# Autodesk Inventor assembly: OT2-Gripper V1-1 BG
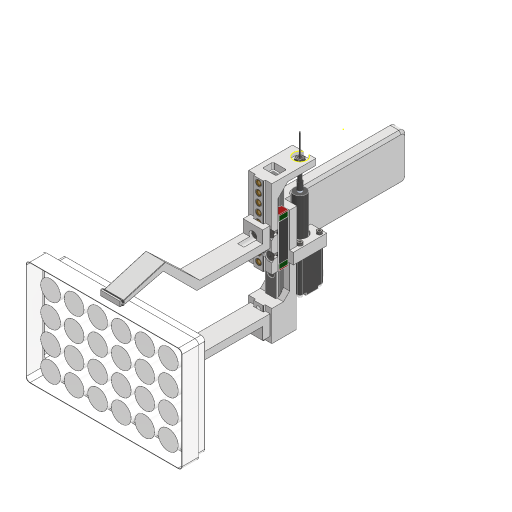
[picture p0: Inventor's stored thumbnail of the model, 512x512]
Saved by Autodesk Inventor 2024.3 (Build 283343000, 343)
## iProperties
Created: 2024-09-13
Part Number: OT2-Gripper V1-1 BG
Document SubType Name: Assembly
Designer: Martin
Author: Martin
## Documents named in this file (15)
- D:\User\Dokumente\GitHub\openUC2-OT2-PlateGripper\INVENTOR\OT2-Gripper V1-1 BG.iam
- D:\User\Dokumente\GitHub\openUC2-OT2-PlateGripper\INVENTOR\OT2-Gripper V1-1 - gripper A.ipt
- D:\User\Dokumente\GitHub\openUC2-OT2-PlateGripper\INVENTOR\OT2-Gripper V1-1 - OT2-interface adapter.ipt
- D:\User\Dokumente\GitHub\openUC2-OT2-PlateGripper\INVENTOR\OT2-Gripper V1-1 - linear adapter static.ipt
- D:\User\Dokumente\GitHub\openUC2-OT2-PlateGripper\INVENTOR\OT2-Gripper V1-1 - linear-adapter.ipt
- D:\User\Dokumente\GitHub\openUC2-OT2-PlateGripper\INVENTOR\00_Joy-IT-B20SHD4353_NEMA8_captive.ipt
- D:\User\Dokumente\GitHub\openUC2-OT2-PlateGripper\INVENTOR\Threaded Insert-Ruthex-M3.ipt
- D:\User\Dokumente\Inventor\Content Center Files\R2024\de-DE\ISO 4032(2)\ISO 4032 - M3 - ISO.ipt
- D:\User\Dokumente\GitHub\openUC2-OT2-PlateGripper\INVENTOR\Actuator_MGN-BG.iam
- D:\User\Dokumente\GitHub\openUC2-OT2-PlateGripper\INVENTOR\00_24wellplate_base_2.ipt
- D:\User\Dokumente\Inventor\Content Center Files\R2024\de-DE\ISO 7091\ISO 7091 - ST 3 - 100 HV.ipt
- D:\User\Dokumente\GitHub\openUC2-OT2-PlateGripper\INVENTOR\o-ring eg MISUMI NSF12.ipt
- D:\User\Dokumente\Inventor\Content Center Files\R2024\de-DE\ISO 4762(2)\ISO 4762 - M2 x 12ISO.ipt
- D:\User\Dokumente\Inventor\Content Center Files\R2024\de-DE\ISO 10642(1)\ISO 10642 - M3 x  8.ipt
- D:\User\Dokumente\Inventor\Content Center Files\R2024\de-DE\ISO 4762(2)\ISO 4762 - M3 x 8ISO.ipt
## Components (44 placed, 14 different names)
1. OT2-Gripper V1-1 - OT2-interface adapter:1 — Einfügen:1, Einfügen:2, Einfügen:3, Passend:1, Passend:3, Passend:9, Einfügen:27, Einfügen:28, Einfügen:29, Einfügen:30, Einfügen:31, Einfügen:32
2. OT2-Gripper V1-1 - linear adapter static:1 — Einfügen:6, Einfügen:7, Einfügen:15, Einfügen:16, Winkel:2, Winkel:3, Passend:2, Passend:8, Winkel:4, Passend:12, Passend:13
3. OT2-Gripper V1-1 - linear-adapter:1 — Einfügen:4, Einfügen:5, Einfügen:8, Einfügen:9, Einfügen:10, Einfügen:11, Einfügen:12, Einfügen:13, Einfügen:14, Passend:4, Passend:5, Passend:6, Passend:7, Passend:10, Passend:11, Passend:14, Einfügen:26
4. OT2-Gripper V1-1 - gripper A:1 — Fluchtend:1, Fluchtend:2, Passend:12, Einfügen:17, Fluchtend:4, Tangential:5, Tangential:6, Tangential:7, Tangential:8, Passend:13
5. OT2-Gripper V1-1 - gripper A:2 — Fluchtend:1, Fluchtend:2, Passend:14, Tangential:1, Tangential:2, Tangential:3, Tangential:4
6. Threaded Insert-Ruthex-M3:14 — Einfügen:29
7. Threaded Insert-Ruthex-M3:15 — Einfügen:27
8. Threaded Insert-Ruthex-M3:16 — Einfügen:28
9. o-ring eg MISUMI NSF12:1 — Tangential:5, Tangential:6, Tangential:7, Tangential:8, Tangential:9
10. o-ring eg MISUMI NSF12:2 — Tangential:1, Tangential:2, Tangential:3, Tangential:4
11. Threaded Insert-Ruthex-M3:1 — Einfügen:3
12. Threaded Insert-Ruthex-M3:2 — Einfügen:4
13. Threaded Insert-Ruthex-M3:3 — Einfügen:5
14. Threaded Insert-Ruthex-M3:4 — Einfügen:2
15. Threaded Insert-Ruthex-M3:5 — Einfügen:14
16. Threaded Insert-Ruthex-M3:6 — Einfügen:13
17. Threaded Insert-Ruthex-M3:7 — Einfügen:12
18. Threaded Insert-Ruthex-M3:8 — Einfügen:11, Einfügen:18
19. Threaded Insert-Ruthex-M3:9 — Einfügen:10
20. Threaded Insert-Ruthex-M3:10 — Einfügen:9
21. Threaded Insert-Ruthex-M3:11 — Einfügen:7
22. Threaded Insert-Ruthex-M3:12 — Einfügen:6
23. Threaded Insert-Ruthex-M3:13 — Einfügen:8
24. 00_Joy-IT-B20SHD4353_NEMA8_captive:1 — Einfügen:1, Winkel:1, Passend:11
25. Actuator_MGN-BG:1 [sub-assembly] — Passend:1, Passend:2, Passend:3, Passend:4, Passend:5, Passend:6, Passend:7, Passend:8, Winkel:4, Passend:9, Passend:10
26. ISO 4762 M2 x 12:1 — Einfügen:30
27. ISO 4762 M2 x 12:2 — Einfügen:31
28. ISO 4762 M2 x 12:3 — Einfügen:32
29. ISO 10642 M3x8:1
30. ISO 10642 M3x8:2
31. ISO 10642 M3x8:3
32. ISO 10642 M3x8:4
33. ISO 4032 M3:3 — Einfügen:25, Einfügen:26
34. ISO 7091 ST 3 - 100 HV:1 — Einfügen:25
35. ISO 4032 M3:1 — Einfügen:16, Winkel:3
36. ISO 4032 M3:2 — Einfügen:15, Winkel:2
37. ISO 4762 M3 x 8:1 — Einfügen:17
38. ISO 4762 M3 x 8:2 — Einfügen:18
39. ISO 4762 M3 x 8:3
40. ISO 4762 M3 x 8:4
41. ISO 4762 M3 x 8:5
42. ISO 4762 M3 x 8:6
43. ISO 4762 M3 x 8:7
44. 00_24wellplate_base_2:1 — Fluchtend:3, Fluchtend:4, Tangential:9
## Relationships (66: Insert 31, Mate 18, Tangent 9, Angle 4, Flush 4)
- Einfügen:1 [Insert]: OT2-Gripper V1-1 - OT2-interface adapter:1 ↔ 00_Joy-IT-B20SHD4353_NEMA8_captive:1
- Winkel:1 [Angle] (180 deg): 00_Joy-IT-B20SHD4353_NEMA8_captive:1
- Einfügen:2 [Insert]: OT2-Gripper V1-1 - OT2-interface adapter:1 ↔ Threaded Insert-Ruthex-M3:4
- Einfügen:3 [Insert]: OT2-Gripper V1-1 - OT2-interface adapter:1 ↔ Threaded Insert-Ruthex-M3:1
- Einfügen:4 [Insert]: OT2-Gripper V1-1 - linear-adapter:1 ↔ Threaded Insert-Ruthex-M3:2
- Einfügen:5 [Insert]: OT2-Gripper V1-1 - linear-adapter:1 ↔ Threaded Insert-Ruthex-M3:3
- Einfügen:6 [Insert]: OT2-Gripper V1-1 - linear adapter static:1 ↔ Threaded Insert-Ruthex-M3:12
- Einfügen:7 [Insert]: OT2-Gripper V1-1 - linear adapter static:1 ↔ Threaded Insert-Ruthex-M3:11
- Einfügen:8 [Insert]: OT2-Gripper V1-1 - linear-adapter:1 ↔ Threaded Insert-Ruthex-M3:13
- Einfügen:9 [Insert]: OT2-Gripper V1-1 - linear-adapter:1 ↔ Threaded Insert-Ruthex-M3:10
- Einfügen:10 [Insert]: OT2-Gripper V1-1 - linear-adapter:1 ↔ Threaded Insert-Ruthex-M3:9
- Einfügen:11 [Insert]: OT2-Gripper V1-1 - linear-adapter:1 ↔ Threaded Insert-Ruthex-M3:8
- Einfügen:12 [Insert]: OT2-Gripper V1-1 - linear-adapter:1 ↔ Threaded Insert-Ruthex-M3:7
- Einfügen:13 [Insert]: OT2-Gripper V1-1 - linear-adapter:1 ↔ Threaded Insert-Ruthex-M3:6
- Einfügen:14 [Insert]: OT2-Gripper V1-1 - linear-adapter:1 ↔ Threaded Insert-Ruthex-M3:5
- Einfügen:15 [Insert]: OT2-Gripper V1-1 - linear adapter static:1 ↔ ISO 4032 M3:2
- Einfügen:16 [Insert]: OT2-Gripper V1-1 - linear adapter static:1 ↔ ISO 4032 M3:1
- Winkel:2 [Angle] (0 deg): OT2-Gripper V1-1 - linear adapter static:1 ↔ ISO 4032 M3:2
- Winkel:3 [Angle] (0 deg): OT2-Gripper V1-1 - linear adapter static:1 ↔ ISO 4032 M3:1
- Passend:1 [Mate]: OT2-Gripper V1-1 - OT2-interface adapter:1 ↔ Actuator_MGN-BG:1
- Passend:2 [Mate]: OT2-Gripper V1-1 - linear adapter static:1 ↔ Actuator_MGN-BG:1
- Passend:3 [Mate]: OT2-Gripper V1-1 - OT2-interface adapter:1 ↔ Actuator_MGN-BG:1
- Passend:4 [Mate]: OT2-Gripper V1-1 - linear-adapter:1 ↔ Actuator_MGN-BG:1
- Passend:5 [Mate]: OT2-Gripper V1-1 - linear-adapter:1 ↔ Actuator_MGN-BG:1
- Passend:6 [Mate]: OT2-Gripper V1-1 - linear-adapter:1 ↔ Actuator_MGN-BG:1
- Passend:7 [Mate]: OT2-Gripper V1-1 - linear-adapter:1 ↔ Actuator_MGN-BG:1
- Passend:8 [Mate]: OT2-Gripper V1-1 - linear adapter static:1 ↔ Actuator_MGN-BG:1
- Winkel:4 [Angle] (180 deg): OT2-Gripper V1-1 - linear adapter static:1 ↔ Actuator_MGN-BG:1
- Passend:9 [Mate]: OT2-Gripper V1-1 - OT2-interface adapter:1 ↔ Actuator_MGN-BG:1
- Passend:10 [Mate]: OT2-Gripper V1-1 - linear-adapter:1 ↔ Actuator_MGN-BG:1
- Passend:11 [Mate]: OT2-Gripper V1-1 - linear-adapter:1 ↔ 00_Joy-IT-B20SHD4353_NEMA8_captive:1
- Fluchtend:1 [Flush]: OT2-Gripper V1-1 - gripper A:1 ↔ OT2-Gripper V1-1 - gripper A:2
- Fluchtend:2 [Flush]: OT2-Gripper V1-1 - gripper A:1 ↔ OT2-Gripper V1-1 - gripper A:2
- Passend:12 [Mate]: OT2-Gripper V1-1 - linear adapter static:1 ↔ OT2-Gripper V1-1 - gripper A:1
- Passend:13 [Mate]: OT2-Gripper V1-1 - linear adapter static:1 ↔ OT2-Gripper V1-1 - gripper A:1
- Passend:14 [Mate]: OT2-Gripper V1-1 - linear-adapter:1 ↔ OT2-Gripper V1-1 - gripper A:2
- Einfügen:17 [Insert]: OT2-Gripper V1-1 - gripper A:1 ↔ ISO 4762 M3 x 8:1
- Einfügen:18 [Insert]: Threaded Insert-Ruthex-M3:8 ↔ ISO 4762 M3 x 8:2
- [Insert]: Actuator_MGN-BG:1 ↔ ISO 4762 M3 x 8:3
- [Insert]: Actuator_MGN-BG:1 ↔ ISO 4762 M3 x 8:4
- [Insert]: Actuator_MGN-BG:1 ↔ ISO 4762 M3 x 8:5
- [Insert]: Actuator_MGN-BG:1 ↔ ISO 4762 M3 x 8:6
- [Insert]: Actuator_MGN-BG:1 ↔ ISO 4762 M3 x 8:7
- Fluchtend:3 [Flush]: 00_24wellplate_base_2:1
- Fluchtend:4 [Flush] (-5 mm): OT2-Gripper V1-1 - gripper A:1 ↔ 00_24wellplate_base_2:1
- Einfügen:25 [Insert]: ISO 4032 M3:3 ↔ ISO 7091 ST 3 - 100 HV:1
- Einfügen:26 [Insert]: OT2-Gripper V1-1 - linear-adapter:1 ↔ ISO 4032 M3:3
- Tangential:1: OT2-Gripper V1-1 - gripper A:2 ↔ o-ring eg MISUMI NSF12:2
- Tangential:2: OT2-Gripper V1-1 - gripper A:2 ↔ o-ring eg MISUMI NSF12:2
- Tangential:3: OT2-Gripper V1-1 - gripper A:2 ↔ o-ring eg MISUMI NSF12:2
- Tangential:4: OT2-Gripper V1-1 - gripper A:2 ↔ o-ring eg MISUMI NSF12:2
- Tangential:5: OT2-Gripper V1-1 - gripper A:1 ↔ o-ring eg MISUMI NSF12:1
- Tangential:6: OT2-Gripper V1-1 - gripper A:1 ↔ o-ring eg MISUMI NSF12:1
- Tangential:7: OT2-Gripper V1-1 - gripper A:1 ↔ o-ring eg MISUMI NSF12:1
- Tangential:8: OT2-Gripper V1-1 - gripper A:1 ↔ o-ring eg MISUMI NSF12:1
- Tangential:9: o-ring eg MISUMI NSF12:1 ↔ 00_24wellplate_base_2:1
- [Mate]: OT2-Gripper V1-1 - linear-adapter:1 ↔ ISO 10642 M3x8:1
- [Mate]: OT2-Gripper V1-1 - linear-adapter:1 ↔ ISO 10642 M3x8:2
- [Mate]: OT2-Gripper V1-1 - linear-adapter:1 ↔ ISO 10642 M3x8:3
- [Mate]: OT2-Gripper V1-1 - linear-adapter:1 ↔ ISO 10642 M3x8:4
- Einfügen:27 [Insert]: OT2-Gripper V1-1 - OT2-interface adapter:1 ↔ Threaded Insert-Ruthex-M3:15
- Einfügen:28 [Insert]: OT2-Gripper V1-1 - OT2-interface adapter:1 ↔ Threaded Insert-Ruthex-M3:16
- Einfügen:29 [Insert]: OT2-Gripper V1-1 - OT2-interface adapter:1 ↔ Threaded Insert-Ruthex-M3:14
- Einfügen:30 [Insert]: OT2-Gripper V1-1 - OT2-interface adapter:1 ↔ ISO 4762 M2 x 12:1
- Einfügen:31 [Insert]: OT2-Gripper V1-1 - OT2-interface adapter:1 ↔ ISO 4762 M2 x 12:2
- Einfügen:32 [Insert]: OT2-Gripper V1-1 - OT2-interface adapter:1 ↔ ISO 4762 M2 x 12:3
